# Autodesk Inventor assembly: 5 Support Compartment Model
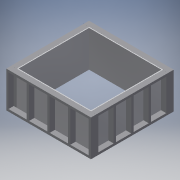
[picture p0: Inventor's stored thumbnail of the model, 180x180]
Saved by Autodesk Inventor 2017 (Build 210142000, 142)
## iProperties
Created: 2017-05-25
Part Number: 5 Support Compartment Model
Document SubType Name: Assembly
Designer: cas7
Author: cas7
## Documents named in this file (4)
- C:\Users\Public\Documents\Autodesk\.desktop-connect\.docstore\guided-tutorial-plugin\INVNTOR\5 Support Compartment Model.iam
- C:\Users\Public\Documents\Autodesk\.desktop-connect\.docstore\guided-tutorial-plugin\INVNTOR\2017\ENU\552100320579484105\TutorialModelPath\4x2 Gyp Board.ipt
- C:\Users\Public\Documents\Autodesk\.desktop-connect\.docstore\guided-tutorial-plugin\INVNTOR\5 Support Model.iam
- C:\Users\Public\Documents\Autodesk\.desktop-connect\.docstore\guided-tutorial-plugin\INVNTOR\Compartment Modeling\Extended 5 compartment frame.iam
## Components (6 placed, 3 different names)
1. 5 Support Model:1 [sub-assembly] — Mate:1, Mate:2, Mate:9
2. 5 Support Model:3 [sub-assembly] — Mate:3, Mate:4, Mate:5, Mate:6, Mate:7
3. Extended 5 compartment frame:1 [sub-assembly] — Mate:5, Mate:6, Mate:10
4. Extended 5 compartment frame:2 [sub-assembly] — Mate:1, Mate:2, Mate:3, Mate:4, Mate:8
5. 4x2 Gyp Board:1 — Mate:7, Mate:8
6. 4x2 Gyp Board:2 — Mate:9, Mate:10
## Relationships (10: Mate 10)
- Mate:1: 5 Support Model:1 ↔ Extended 5 compartment frame:2
- Mate:2: 5 Support Model:1 ↔ Extended 5 compartment frame:2
- Mate:3: 5 Support Model:3 ↔ Extended 5 compartment frame:2
- Mate:4: 5 Support Model:3 ↔ Extended 5 compartment frame:2
- Mate:5: 5 Support Model:3 ↔ Extended 5 compartment frame:1
- Mate:6: 5 Support Model:3 ↔ Extended 5 compartment frame:1
- Mate:7: 5 Support Model:3 ↔ 4x2 Gyp Board:1
- Mate:8: Extended 5 compartment frame:2 ↔ 4x2 Gyp Board:1
- Mate:9: 5 Support Model:1 ↔ 4x2 Gyp Board:2
- Mate:10: Extended 5 compartment frame:1 ↔ 4x2 Gyp Board:2
